# Autodesk Inventor assembly: каретка
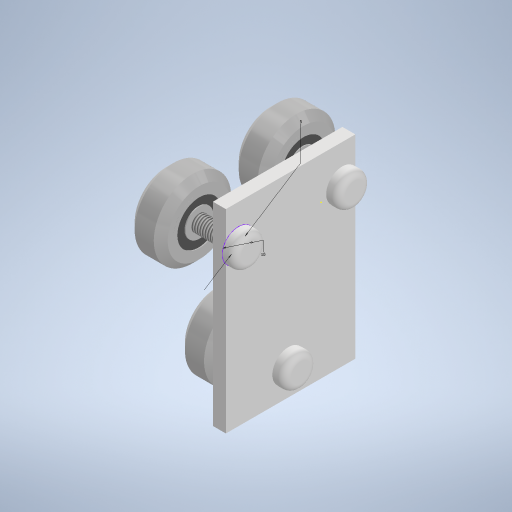
[picture p0: Inventor's stored thumbnail of the model, 512x512]
Saved by Autodesk Inventor 2024.2 (Build 282272000, 272)
## iProperties
Created: 2026-01-30
Part Number: каретка
Document SubType Name: Assembly
Designer: Service
Author: Service
## Documents named in this file (4)
- C:\Users\Service\Documents\Artist-v2\3D\каретка.iam
- C:\Users\Service\Documents\Основание.ipt
- C:\Users\Service\Documents\м5.ipt
- C:\Users\Service\Documents\колесико.iam
## Components (7 placed, 3 different names)
1. Основание:1 — Заподлицо:1, Заподлицо:2, Совмещение:1, Совмещение:2, Совмещение:3, Совмещение:4, Совмещение:5, Совмещение:7, Совмещение:10, Совмещение:11
2. м5:1 — Заподлицо:1, Заподлицо:2, Совмещение:1, Совмещение:8
3. м5:2 — Совмещение:3, Совмещение:4, Совмещение:6
4. м5:3 — Совмещение:2, Совмещение:5, Совмещение:9
5. колесико:2 [sub-assembly] — Совмещение:6, Совмещение:7
6. колесико:3 [sub-assembly] — Совмещение:8, Совмещение:10
7. колесико:4 [sub-assembly] — Совмещение:9, Совмещение:11
## Relationships (13: Mate 11, Flush 2)
- Заподлицо:1 [Flush]: Основание:1 ↔ м5:1
- Заподлицо:2 [Flush]: Основание:1 ↔ м5:1
- Совмещение:1 [Mate]: Основание:1 ↔ м5:1
- Совмещение:2 [Mate]: Основание:1 ↔ м5:3
- Совмещение:3 [Mate]: Основание:1 ↔ м5:2
- Совмещение:4 [Mate]: Основание:1 ↔ м5:2
- Совмещение:5 [Mate]: Основание:1 ↔ м5:3
- Совмещение:6 [Mate]: м5:2 ↔ колесико:2
- Совмещение:7 [Mate] (8 mm): Основание:1 ↔ колесико:2
- Совмещение:8 [Mate]: м5:1 ↔ колесико:3
- Совмещение:9 [Mate]: м5:3 ↔ колесико:4
- Совмещение:10 [Mate] (8 mm): Основание:1 ↔ колесико:3
- Совмещение:11 [Mate] (8 mm): Основание:1 ↔ колесико:4
